# Autodesk Inventor assembly: UpperArm
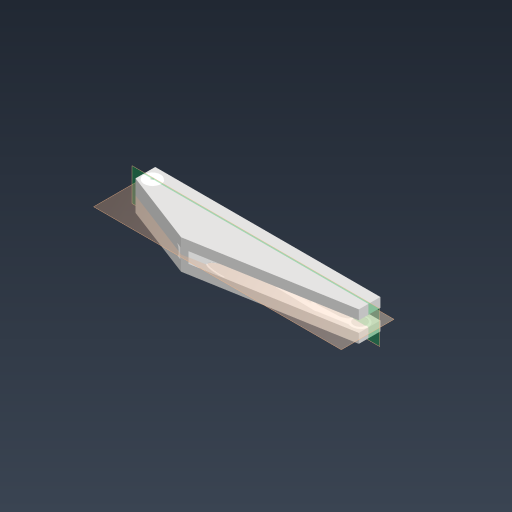
[picture p0: Inventor's stored thumbnail of the model, 512x512]
Saved by Autodesk Inventor 2023 (Build 270158000, 158)
## iProperties
Created: 2023-03-17
Part Number: UpperArm
Document SubType Name: Assembly
Designer: valer
Author: valer
## Documents named in this file (3)
- C:\Users\valer\Desktop\str1ker\cad\UpperArm.iam
- C:\Users\valer\Desktop\str1ker\cad\UpperArm.ipt
- C:\Users\valer\Desktop\str1ker\cad\UpperArmBoundingBox.ipt
## Components (2 placed, 2 different names)
1. UpperArm:1 — Mate:1, Angle:1, Angle:2
2. UpperArmBoundingBox:1 — Mate:2, Angle:3, Angle:4
## Relationships (6: Angle 4, Mate 2)
- Mate:1: UpperArm:1
- Angle:1 (270 deg): UpperArm:1
- Angle:2 (0 deg): UpperArm:1
- Mate:2: UpperArmBoundingBox:1
- Angle:3 (0 deg): UpperArmBoundingBox:1
- Angle:4 (0 deg): UpperArmBoundingBox:1
